# Autodesk Inventor assembly: GE-20020_Vinyl Red_Axle
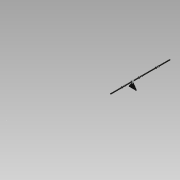
[picture p0: Inventor's stored thumbnail of the model, 180x180]
Saved by Autodesk Inventor 2020.1 (Build 241239000, 239)
## iProperties
Created: 2019-10-14
Part Number: GE-20020_Vinyl Red_Axle
Document SubType Name: Assembly
Designer: Phillips Lenovo
Author: Phillips Lenovo
Revision Number: ANY
## Documents named in this file (12)
- D:\FIRST 2020\FRC 2020\FRC Field 2020\Parts\GE-20020_Vinyl Red_Axle.iam
- D:\FIRST 2020\FRC 2020\FRC Field 2020\Parts\pin_clevis_.25_1.75_pin_clevis_.25_1.75.ipt
- D:\FIRST 2020\FRC 2020\FRC Field 2020\Parts\pin_cotter_.0625_.50_pin_cotter_.0625_.50.ipt
- D:\FIRST 2020\FRC 2020\FRC Field 2020\Parts\hex_.5_20_1.75_92865A732.ipt
- D:\FIRST 2020\FRC 2020\FRC Field 2020\Parts\washer_flat_.5_98023A029.ipt
- D:\FIRST 2020\FRC 2020\FRC Field 2020\Parts\nylock_.50_20_95615A220.ipt
- D:\FIRST 2020\FRC 2020\FRC Field 2020\Parts\GE-20015.ipt
- D:\FIRST 2020\FRC 2020\FRC Field 2020\Parts\6435K230_ONE-PIECE CLAMP-ON SHAFT COLLAR_6435K23.ipt
- D:\FIRST 2020\FRC 2020\FRC Field 2020\Parts\GE-20013.ipt
- D:\FIRST 2020\FRC 2020\FRC Field 2020\Parts\3126T310_RAILING CLAMP_KC_3126T31.ipt
- D:\FIRST 2020\FRC 2020\FRC Field 2020\Parts\hanger sensor.ipt
- D:\FIRST 2020\FRC 2020\FRC Field 2020\Parts\GE-20014.ipt
## Components (33 placed, 33 different names)
1. GE-20015_1019 — Flush:1
2. GE-20015_1020
3. GE-20015_1021
4. GE-20015_1022
5. GE-20015_1023
6. GE-20015_1024
7. 6435K230_ONE-PIECE CLAMP-ON SHAFT COLLAR_6435K23_1025
8. 6435K230_ONE-PIECE CLAMP-ON SHAFT COLLAR_6435K23_1026
9. 6435K230_ONE-PIECE CLAMP-ON SHAFT COLLAR_6435K23_1027
10. 6435K230_ONE-PIECE CLAMP-ON SHAFT COLLAR_6435K23_1028
11. 6435K230_ONE-PIECE CLAMP-ON SHAFT COLLAR_6435K23_1029
12. 6435K230_ONE-PIECE CLAMP-ON SHAFT COLLAR_6435K23_1030
13. GE-20013_1031
14. 3126T310_RAILING CLAMP_KC_3126T31_1071
15. hanger sensor_1072
16. hanger sensor_1073
17. GE-20014_1074
18. pin_clevis_.25_1.75_pin_clevis_.25_1.75_998
19. pin_cotter_.0625_.50_pin_cotter_.0625_.50_999
20. hex_.5_20_1.75_92865A732_1000
21. washer_flat_.5_98023A029_1001
22. nylock_.50_20_95615A220_1002
23. pin_cotter_.0625_.50_pin_cotter_.0625_.50_1065
24. pin_clevis_.25_1.75_pin_clevis_.25_1.75_1066
25. pin_cotter_.0625_.50_pin_cotter_.0625_.50_1067
26. pin_cotter_.0625_.50_pin_cotter_.0625_.50_1068
27. pin_clevis_.25_1.75_pin_clevis_.25_1.75_1069
28. pin_clevis_.25_1.75_pin_clevis_.25_1.75_1070
29. pin_cotter_.0625_.50_pin_cotter_.0625_.50_1075
30. pin_cotter_.0625_.50_pin_cotter_.0625_.50_1076
31. pin_clevis_.25_1.75_pin_clevis_.25_1.75_1077
32. pin_clevis_.25_1.75_pin_clevis_.25_1.75_1078
33. pin_cotter_.0625_.50_pin_cotter_.0625_.50:7
## Relationships (3: Mate 2, Flush 1)
- Flush:1 (25.4889 mm): GE-20015_1019
- Mate:2
- Mate:8
